# Autodesk Inventor assembly: BeltDriveTest
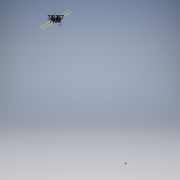
[picture p0: Inventor's stored thumbnail of the model, 180x180]
Saved by Autodesk Inventor 2018.3 (Build 223284000, 284)
## iProperties
Created: 2018-07-29
Part Number: BeltDriveTest
Material: Generisch
Document SubType Name: Assembly
Designer: JochenAlt
Author: JochenAlt
## Documents named in this file (5)
- D:\Projects\Ondine\CAD\Beltdrive\BeltDriveTestBed.iam
- D:\Projects\Ondine\CAD\Beltdrive\BeltDriveConstruction.iam
- D:\Projects\Ondine\CAD\Beltdrive\BeltDriveTestHolder.ipt
- D:\Projects\Ondine\CAD\Mounting Hub.ipt
- D:\Projects\Ondine\CAD\Beltdrive\ZwischenScheibe.ipt
## Components (5 placed, 4 different names)
1. BeltDriveConstruction:1 [sub-assembly] — Passend:1, Passend:3, Passend:13, Fluchtend:1, Passend:14, Passend:15, Passend:17
2. BeltDriveTestHolder:1 — Passend:3, Passend:9, Passend:12
3. BeltDriveTestHolder:2 — Passend:1, Passend:12, Passend:16
4. Mounting Hub:1 — Passend:9
5. Synchrone Riemenscheibe1:1 — Passend:13, Fluchtend:1
## Relationships (10: Mate 9, Flush 1)
- Passend:1 [Mate]: BeltDriveConstruction:1 ↔ BeltDriveTestHolder:2
- Passend:3 [Mate]: BeltDriveConstruction:1 ↔ BeltDriveTestHolder:1
- Passend:9 [Mate] (1 mm): BeltDriveTestHolder:1 ↔ Mounting Hub:1
- Passend:12 [Mate]: BeltDriveTestHolder:1 ↔ BeltDriveTestHolder:2
- Passend:13 [Mate]: BeltDriveConstruction:1 ↔ Synchrone Riemenscheibe1:1
- Fluchtend:1 [Flush] (0.5 mm): BeltDriveConstruction:1 ↔ Synchrone Riemenscheibe1:1
- Passend:14 [Mate]: BeltDriveConstruction:1
- Passend:15 [Mate]: BeltDriveConstruction:1
- Passend:16 [Mate]: BeltDriveTestHolder:2
- Passend:17 [Mate]: BeltDriveConstruction:1
